# Autodesk Inventor assembly: BIKE V-BRAKE
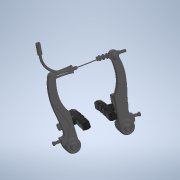
[picture p0: Inventor's stored thumbnail of the model, 180x180]
Saved by Autodesk Inventor 2021 (Build 250183000, 183)
## iProperties
Created: 2011-10-28
Part Number: BIKE V-BRAKE
Description: STEP AP203
Document SubType Name: Assembly
Designer: j2seb
Sending System: SolidWorks 2011
Preprocessor: SwSTEP 2.0
Title: BIKE V-BRAKE.STEP
Revision Number: ANY
## Documents named in this file (35)
- C:\Git\Proyecto_APM\02 Inventor\bicicleta_ruta\Freno\BIKE V-BRAKE.iam
- C:\Git\Proyecto_APM\02 Inventor\bicicleta_ruta\Freno\001162-26.ipt
- C:\Git\Proyecto_APM\02 Inventor\bicicleta_ruta\Freno\001162-22.ipt
- C:\Git\Proyecto_APM\02 Inventor\bicicleta_ruta\Freno\001162-18.ipt
- C:\Git\Proyecto_APM\02 Inventor\bicicleta_ruta\Freno\001162-34.ipt
- C:\Git\Proyecto_APM\02 Inventor\bicicleta_ruta\Freno\001162-31.ipt
- C:\Git\Proyecto_APM\02 Inventor\bicicleta_ruta\Freno\001162-30.ipt
- C:\Git\Proyecto_APM\02 Inventor\bicicleta_ruta\Freno\001162-25.ipt
- C:\Git\Proyecto_APM\02 Inventor\bicicleta_ruta\Freno\001162-17.ipt
- C:\Git\Proyecto_APM\02 Inventor\bicicleta_ruta\Freno\001162-29.ipt
- C:\Git\Proyecto_APM\02 Inventor\bicicleta_ruta\Freno\001162-24.ipt
- C:\Git\Proyecto_APM\02 Inventor\bicicleta_ruta\Freno\001162-20.ipt
- C:\Git\Proyecto_APM\02 Inventor\bicicleta_ruta\Freno\001162-16.ipt
- C:\Git\Proyecto_APM\02 Inventor\bicicleta_ruta\Freno\001162-35.ipt
- C:\Git\Proyecto_APM\02 Inventor\bicicleta_ruta\Freno\001162-27.ipt
- C:\Git\Proyecto_APM\02 Inventor\bicicleta_ruta\Freno\001162-15.ipt
- C:\Git\Proyecto_APM\02 Inventor\bicicleta_ruta\Freno\001162-21.ipt
- C:\Git\Proyecto_APM\02 Inventor\bicicleta_ruta\Freno\001162-10.ipt
- C:\Git\Proyecto_APM\02 Inventor\bicicleta_ruta\Freno\001162-32.ipt
- C:\Git\Proyecto_APM\02 Inventor\bicicleta_ruta\Freno\001162-23.ipt
- C:\Git\Proyecto_APM\02 Inventor\bicicleta_ruta\Freno\001162-14.ipt
- C:\Git\Proyecto_APM\02 Inventor\bicicleta_ruta\Freno\001162-9.ipt
- C:\Git\Proyecto_APM\02 Inventor\bicicleta_ruta\Freno\001162-19.ipt
- C:\Git\Proyecto_APM\02 Inventor\bicicleta_ruta\Freno\001162-8.ipt
- C:\Git\Proyecto_APM\02 Inventor\bicicleta_ruta\Freno\001162-5.ipt
- C:\Git\Proyecto_APM\02 Inventor\bicicleta_ruta\Freno\001162-4.ipt
- C:\Git\Proyecto_APM\02 Inventor\bicicleta_ruta\Freno\001162-13.ipt
- C:\Git\Proyecto_APM\02 Inventor\bicicleta_ruta\Freno\001162-12.ipt
- C:\Git\Proyecto_APM\02 Inventor\bicicleta_ruta\Freno\001162-11.ipt
- C:\Git\Proyecto_APM\02 Inventor\bicicleta_ruta\Freno\001162-7.ipt
- C:\Git\Proyecto_APM\02 Inventor\bicicleta_ruta\Freno\001162-6.ipt
- C:\Git\Proyecto_APM\02 Inventor\bicicleta_ruta\Freno\001162-3.ipt
- C:\Git\Proyecto_APM\02 Inventor\bicicleta_ruta\Freno\001162-2.ipt
- C:\Git\Proyecto_APM\02 Inventor\bicicleta_ruta\Freno\001162-28.ipt
- C:\Git\Proyecto_APM\02 Inventor\bicicleta_ruta\Freno\001162-1.ipt
## Components (36 placed, 36 different names)
1. 001162-26_1
2. 001162-22_2
3. 001162-18_3
4. 001162-34_4 — Mate:2
5. 001162-31_5
6. 001162-30_6
7. 001162-25_7
8. 001162-17_8
9. 001162-29_9
10. 001162-24_10
11. 001162-20_11
12. 001162-16_12
13. 001162-35_13
14. 001162-27_14
15. 001162-15_15
16. 001162-21_16
17. 001162-10_17
18. 001162-32_18
19. 001162-23_19
20. 001162-14_20
21. 001162-9_21
22. 001162-19_22
23. 001162-8_23
24. 001162-5_24
25. 001162-4_25
26. 001162-13_26
27. 001162-34_27 — Mate:1
28. 001162-12_28
29. 001162-11_29 — Mate:4, Mate:6
30. 001162-7_30 — Mate:3
31. 001162-6_31 — Mate:3
32. 001162-3_32
33. 001162-2_33
34. 001162-28_34
35. 001162-1_35
36. 001162-35_36
## Relationships (9: Mate 8, Angle 1)
- Mate:1: 001162-34_27
- Mate:2: 001162-34_4
- Mate:3: 001162-7_30 ↔ 001162-6_31
- Mate:4: 001162-11_29
- Mate:5
- Mate:6: 001162-11_29
- Mate:7
- Mate:8
- Angle:1 (0 deg)
